# Autodesk Inventor assembly: artschallenge2022
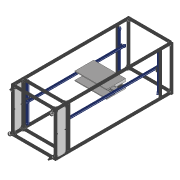
[picture p0: Inventor's stored thumbnail of the model, 180x180]
Saved by Autodesk Inventor 2020 (Build 240168000, 168)
## iProperties
Created: 2021-10-24
Part Number: artschallenge2022
Description: CAx-IF Rec.Pracs.---Model Styling and Organization---1.2---2011-12-15
Document SubType Name: Assembly
Designer: ken113
Sending System: 3D_Kernel_IO2017 Sp2 by CT CoreTechnologie
Preprocessor: STEP Interface 2017 Sp2 by CT CoreTechnologie
Title: artschallenge2022.stp
## Documents named in this file (61)
- D:\Document\Github\Eto_Project\Hardware\Parts\MISUMI_FRAMES\model_ver2\artschallenge2022.iam
- D:\Document\Github\Eto_Project\Hardware\Parts\MISUMI_FRAMES\model_ver2\NEFSB8-4040-200.ipt
- D:\Document\Github\Eto_Project\Hardware\Parts\MISUMI_FRAMES\model_ver2\NEFSB8-4040-1030.ipt
- D:\Document\Github\Eto_Project\Hardware\Parts\MISUMI_FRAMES\model_ver2\NEFSB8-4040-950.ipt
- D:\Document\Github\Eto_Project\Hardware\Parts\MISUMI_FRAMES\model_ver2\HBLFSNB8-C-SET(1).iam
- D:\Document\Github\Eto_Project\Hardware\Parts\MISUMI_FRAMES\model_ver2\HBLFSNB8-C-SET(2).iam
- D:\Document\Github\Eto_Project\Hardware\Parts\MISUMI_FRAMES\model_ver2\HBLFSNB8-C-SET(3).iam
- D:\Document\Github\Eto_Project\Hardware\Parts\MISUMI_FRAMES\model_ver2\HBLFSNB8-C-SET(4).iam
- D:\Document\Github\Eto_Project\Hardware\Parts\MISUMI_FRAMES\model_ver2\HBLFSNB8-SET(1).iam
- D:\Document\Github\Eto_Project\Hardware\Parts\MISUMI_FRAMES\model_ver2\HBLFSNB8-SET(2).iam
- D:\Document\Github\Eto_Project\Hardware\Parts\MISUMI_FRAMES\model_ver2\HBLFSNB8-SET(3).iam
- D:\Document\Github\Eto_Project\Hardware\Parts\MISUMI_FRAMES\model_ver2\HBLFSNB8-SET(4).iam
- D:\Document\Github\Eto_Project\Hardware\Parts\MISUMI_FRAMES\model_ver2\HBLFSNB8-SET(5).iam
- D:\Document\Github\Eto_Project\Hardware\Parts\MISUMI_FRAMES\model_ver2\HBLFSNB8-SET(6).iam
- D:\Document\Github\Eto_Project\Hardware\Parts\MISUMI_FRAMES\model_ver2\HBLFSNB8-SET(7).iam
- D:\Document\Github\Eto_Project\Hardware\Parts\MISUMI_FRAMES\model_ver2\HBLFSNB8-SET(8).iam
- D:\Document\Github\Eto_Project\Hardware\Parts\MISUMI_FRAMES\model_ver2\HBLFSNB8-C-SET(5).iam
- D:\Document\Github\Eto_Project\Hardware\Parts\MISUMI_FRAMES\model_ver2\HBLFSNB8-C-SET(6).iam
- D:\Document\Github\Eto_Project\Hardware\Parts\MISUMI_FRAMES\model_ver2\HBLFSNB8-SET(9).iam
- D:\Document\Github\Eto_Project\Hardware\Parts\MISUMI_FRAMES\model_ver2\HBLFSNB8-SET(10).iam
- D:\Document\Github\Eto_Project\Hardware\Parts\MISUMI_FRAMES\model_ver2\HBLFSNB8-SET(11).iam
- D:\Document\Github\Eto_Project\Hardware\Parts\MISUMI_FRAMES\model_ver2\HBLFSNB8-SET(12).iam
- D:\Document\Github\Eto_Project\Hardware\Parts\MISUMI_FRAMES\model_ver2\HBLFSNB8-SET(13).iam
- D:\Document\Github\Eto_Project\Hardware\Parts\MISUMI_FRAMES\model_ver2\HBLFSNB8-SET(14).iam
- D:\Document\Github\Eto_Project\Hardware\Parts\MISUMI_FRAMES\model_ver2\HBLFSNB8-SET(15).iam
- D:\Document\Github\Eto_Project\Hardware\Parts\MISUMI_FRAMES\model_ver2\HBLFSNB8-SET(16).iam
- D:\Document\Github\Eto_Project\Hardware\Parts\MISUMI_FRAMES\model_ver2\HBLFSNB8-C-SET(7).iam
- D:\Document\Github\Eto_Project\Hardware\Parts\MISUMI_FRAMES\model_ver2\HBLFSNB8-C-SET(8).iam
- D:\Document\Github\Eto_Project\Hardware\Parts\MISUMI_FRAMES\model_ver2\NEFSB8-4040-2400.ipt
- D:\Document\Github\Eto_Project\Hardware\Parts\MISUMI_FRAMES\model_ver2\ACBA6H-948-198-3-F463-G176-N5.ipt
- D:\Document\Github\Eto_Project\Hardware\Parts\MISUMI_FRAMES\model_ver2\HSMCS75-R.iam
- D:\Document\Github\Eto_Project\Hardware\Parts\MISUMI_FRAMES\model_ver2\HBLFSNB8-SET(17).iam
- D:\Document\Github\Eto_Project\Hardware\Parts\MISUMI_FRAMES\model_ver2\HBLFSNB8-SET(18).iam
- D:\Document\Github\Eto_Project\Hardware\Parts\MISUMI_FRAMES\model_ver2\HBLFSNB8-SET(19).iam
- D:\Document\Github\Eto_Project\Hardware\Parts\MISUMI_FRAMES\model_ver2\HBLFSNB8-SET(20).iam
- D:\Document\Github\Eto_Project\Hardware\Parts\MISUMI_FRAMES\model_ver2\HBLFSNB8-SET(21).iam
- D:\Document\Github\Eto_Project\Hardware\Parts\MISUMI_FRAMES\model_ver2\HBLFSNB8-SET(22).iam
- D:\Document\Github\Eto_Project\Hardware\Parts\MISUMI_FRAMES\model_ver2\HBLFSNB8-SET(23).iam
- D:\Document\Github\Eto_Project\Hardware\Parts\MISUMI_FRAMES\model_ver2\HBLFSNB8-SET(24).iam
- D:\Document\Github\Eto_Project\Hardware\Parts\MISUMI_FRAMES\model_ver2\HBLFSNB8-SET(25).iam
- D:\Document\Github\Eto_Project\Hardware\Parts\MISUMI_FRAMES\model_ver2\HBLFSNB8-SET(26).iam
- D:\Document\Github\Eto_Project\Hardware\Parts\MISUMI_FRAMES\model_ver2\HBLFSNB8-SET(27).iam
- D:\Document\Github\Eto_Project\Hardware\Parts\MISUMI_FRAMES\model_ver2\HBLFSNB8-SET(28).iam
- D:\Document\Github\Eto_Project\Hardware\Parts\MISUMI_FRAMES\model_ver2\HBLFSNB8-SET(29).iam
- D:\Document\Github\Eto_Project\Hardware\Parts\MISUMI_FRAMES\model_ver2\HBLFSNB8-SET(30).iam
- D:\Document\Github\Eto_Project\Hardware\Parts\MISUMI_FRAMES\model_ver2\HBLFSNB8-SET(31).iam
- D:\Document\Github\Eto_Project\Hardware\Parts\MISUMI_FRAMES\model_ver2\HBLFSNB8-SET(32).iam
- D:\Document\Github\Eto_Project\Hardware\Parts\MISUMI_FRAMES\model_ver2\HBLFSNB8-SET(33).iam
- D:\Document\Github\Eto_Project\Hardware\Parts\MISUMI_FRAMES\model_ver2\HBLFSNB8-SET(34).iam
- D:\Document\Github\Eto_Project\Hardware\Parts\MISUMI_FRAMES\model_ver2\HBLFSNB8-SET(35).iam
- D:\Document\Github\Eto_Project\Hardware\Parts\MISUMI_FRAMES\model_ver2\HBLFSNB8-SET(36).iam
- D:\Document\Github\Eto_Project\Hardware\Parts\MISUMI_FRAMES\model_ver2\HCBM5-8.ipt
- D:\Document\Github\Eto_Project\Hardware\Parts\MISUMI_FRAMES\model_ver2\HCBR8.ipt
- D:\Document\Github\Eto_Project\Hardware\Parts\MISUMI_FRAMES\model_ver2\HNTT8-8.ipt
- D:\Document\Github\Eto_Project\Hardware\Parts\MISUMI_FRAMES\model_ver2\CBM8-12.ipt
- D:\Document\Github\Eto_Project\Hardware\Parts\MISUMI_FRAMES\model_ver2\HCBM5-15.ipt
- D:\Document\Github\Eto_Project\Hardware\Parts\CCM\CCM motion linear guide rail\CCM_UNIT\CCM_Unit_A.iam
- D:\Document\Github\Eto_Project\Hardware\Parts\CCM\CCM motion linear guide rail\CCM_UNIT\CCM_Unit_B.iam
- D:\Document\Github\Eto_Project\Hardware\Parts\CCM\CCM motion linear guide rail\CCM_UNIT\CCM_Unit_C.iam
- D:\Document\Github\Eto_Project\Hardware\Parts\CCM\CCM motion linear guide rail\CCM_UNIT\CCM_Unit_D.iam
- D:\Document\Github\Eto_Project\Hardware\Parts\Display\Display_A.ipt
## Components (130 placed, 60 different names)
1. NEFSB8-4040-200
2. NEFSB8-4040-200:1
3. NEFSB8-4040-200:2
4. NEFSB8-4040-200:3
5. NEFSB8-4040-1030
6. NEFSB8-4040-1030:1 — メイト:4, メイト:5
7. NEFSB8-4040-950
8. NEFSB8-4040-950:1
9. HBLFSNB8-C-SET(1) [sub-assembly]
10. HBLFSNB8-C-SET(2) [sub-assembly]
11. HBLFSNB8-C-SET(3) [sub-assembly]
12. HBLFSNB8-C-SET(4) [sub-assembly]
13. HBLFSNB8-SET(1) [sub-assembly]
14. HBLFSNB8-SET(2) [sub-assembly]
15. HBLFSNB8-SET(3) [sub-assembly]
16. HBLFSNB8-SET(4) [sub-assembly]
17. HBLFSNB8-SET(5) [sub-assembly]
18. HBLFSNB8-SET(6) [sub-assembly]
19. HBLFSNB8-SET(7) [sub-assembly]
20. HBLFSNB8-SET(8) [sub-assembly]
21. NEFSB8-4040-1030:2
22. NEFSB8-4040-950:2
23. NEFSB8-4040-950:3
24. NEFSB8-4040-1030:3
25. HBLFSNB8-C-SET(5) [sub-assembly]
26. HBLFSNB8-C-SET(6) [sub-assembly]
27. HBLFSNB8-SET(9) [sub-assembly]
28. HBLFSNB8-SET(10) [sub-assembly]
29. HBLFSNB8-SET(11) [sub-assembly]
30. HBLFSNB8-SET(12) [sub-assembly]
31. HBLFSNB8-SET(13) [sub-assembly]
32. HBLFSNB8-SET(14) [sub-assembly]
33. HBLFSNB8-SET(15) [sub-assembly]
34. HBLFSNB8-SET(16) [sub-assembly]
35. HBLFSNB8-C-SET(7) [sub-assembly]
36. HBLFSNB8-C-SET(8) [sub-assembly]
37. NEFSB8-4040-2400 — メイト:2, メイト:15, フラッシュ:17, メイト:16, フラッシュ:19
38. NEFSB8-4040-2400:1 — 角度:2, メイト:3
39. NEFSB8-4040-2400:2 — 角度:1, メイト:1, メイト:6, メイト:13, フラッシュ:14, メイト:14
40. NEFSB8-4040-2400:3 — 角度:3
41. NEFSB8-4040-1030:4
42. NEFSB8-4040-1030:5 — 角度:4
43. ACBA6H-948-198-3-F463-G176-N5
44. ACBA6H-948-198-3-F463-G176-N5:1
45. HSMCS75-R [sub-assembly]
46. HSMCS75-R:1 [sub-assembly]
47. HSMCS75-R:2 [sub-assembly]
48. HSMCS75-R:3 [sub-assembly]
49. HBLFSNB8-SET(17) [sub-assembly]
50. HBLFSNB8-SET(18) [sub-assembly]
51. HBLFSNB8-SET(19) [sub-assembly]
52. HBLFSNB8-SET(20) [sub-assembly]
53. HBLFSNB8-SET(21) [sub-assembly]
54. HBLFSNB8-SET(22) [sub-assembly]
55. HBLFSNB8-SET(23) [sub-assembly]
56. HBLFSNB8-SET(24) [sub-assembly]
57. HBLFSNB8-SET(25) [sub-assembly]
58. HBLFSNB8-SET(26) [sub-assembly]
59. HBLFSNB8-SET(27) [sub-assembly]
60. HBLFSNB8-SET(28) [sub-assembly]
61. HBLFSNB8-SET(29) [sub-assembly]
62. HBLFSNB8-SET(30) [sub-assembly]
63. HBLFSNB8-SET(31) [sub-assembly]
64. HBLFSNB8-SET(32) [sub-assembly]
65. HBLFSNB8-SET(33) [sub-assembly]
66. HBLFSNB8-SET(34) [sub-assembly]
67. HBLFSNB8-SET(35) [sub-assembly]
68. HBLFSNB8-SET(36) [sub-assembly]
69. NEFSB8-4040-950:4
70. NEFSB8-4040-950:5
71. HCBM5-8
72. HCBM5-8:1
73. HCBM5-8:2
74. HCBM5-8:3
75. HCBR8
76. HCBR8:1
77. HCBM5-8:4
78. HCBM5-8:5
79. HCBM5-8:6
80. HCBM5-8:7
81. HCBR8:2
82. HCBR8:3
83. HNTT8-8
84. CBM8-12
85. HNTT8-8:1
86. CBM8-12:1
87. HNTT8-8:2
88. CBM8-12:2
89. HNTT8-8:3
90. CBM8-12:3
91. HNTT8-8:4
92. CBM8-12:4
93. HNTT8-8:5
94. CBM8-12:5
95. HNTT8-8:6
96. CBM8-12:6
97. HNTT8-8:7
98. CBM8-12:7
99. HNTT8-8:8
100. CBM8-12:8
101. HNTT8-8:9
102. CBM8-12:9
103. HNTT8-8:10
104. CBM8-12:10
105. HNTT8-8:11
106. CBM8-12:11
107. HNTT8-8:12
108. CBM8-12:12
109. HNTT8-8:13
110. CBM8-12:13
111. HNTT8-8:14
112. CBM8-12:14
113. HNTT8-8:15
114. CBM8-12:15
115. HCBM5-15
116. HCBM5-15:1
117. HCBM5-15:2
118. HCBM5-15:3
119. CCM_Unit_A:1 [sub-assembly] — 角度:2, フラッシュ:1, フラッシュ:2, メイト:7, メイト:8, フラッシュ:8, メイト:9, フラッシュ:10, メイト:12, メイト:17
120. CCM_Unit_B:1 [sub-assembly] — 角度:1, 角度:3, フラッシュ:1, フラッシュ:2, メイト:10, フラッシュ:10, メイト:11, フラッシュ:12
121. CCM_Unit_C:1 [sub-assembly] — メイト:1, フラッシュ:3, フラッシュ:5, メイト:6, フラッシュ:6, メイト:9, フラッシュ:16
122. CCM_Unit_C:2 [sub-assembly] — メイト:2, 角度:4, フラッシュ:4, フラッシュ:7, フラッシュ:9, メイト:10
123. CCM_Unit_D:1 [sub-assembly] — メイト:4, フラッシュ:3, フラッシュ:5, メイト:5
124. CCM_Unit_D:2 [sub-assembly] — メイト:3, フラッシュ:4, フラッシュ:6, フラッシュ:7, メイト:7, メイト:8, フラッシュ:8, フラッシュ:9, フラッシュ:15
125. Display_A:1 — 角度:5, フラッシュ:11, メイト:11, フラッシュ:13
126. Display_A:2 — 角度:5, フラッシュ:11, メイト:12, フラッシュ:12, フラッシュ:13, メイト:17
127. NEFSB8-4040-950:7 — メイト:13, フラッシュ:14, フラッシュ:15, フラッシュ:20
128. NEFSB8-4040-950:8 — メイト:16, フラッシュ:19, フラッシュ:20
129. NEFSB8-4040-950:9 — メイト:15, フラッシュ:17, フラッシュ:18
130. NEFSB8-4040-950:10 — メイト:14, フラッシュ:16, フラッシュ:18
## Relationships (42: Flush 20, Mate 17, Angle 5)
- 角度:1 [Angle] (0 deg): NEFSB8-4040-2400:2 ↔ CCM_Unit_B:1
- 角度:2 [Angle] (180 deg): NEFSB8-4040-2400:1 ↔ CCM_Unit_A:1
- 角度:3 [Angle] (0 deg): NEFSB8-4040-2400:3 ↔ CCM_Unit_B:1
- フラッシュ:1 [Flush]: CCM_Unit_A:1 ↔ CCM_Unit_B:1
- フラッシュ:2 [Flush]: CCM_Unit_A:1 ↔ CCM_Unit_B:1
- メイト:1 [Mate] (2 mm): NEFSB8-4040-2400:2 ↔ CCM_Unit_C:1
- メイト:2 [Mate] (2 mm): NEFSB8-4040-2400 ↔ CCM_Unit_C:2
- 角度:4 [Angle] (0 deg): NEFSB8-4040-1030:5 ↔ CCM_Unit_C:2
- メイト:3 [Mate] (2 mm): NEFSB8-4040-2400:1 ↔ CCM_Unit_D:2
- メイト:4 [Mate] (2 mm): NEFSB8-4040-1030:1 ↔ CCM_Unit_D:1
- フラッシュ:3 [Flush]: CCM_Unit_C:1 ↔ CCM_Unit_D:1
- フラッシュ:4 [Flush]: CCM_Unit_C:2 ↔ CCM_Unit_D:2
- フラッシュ:5 [Flush]: CCM_Unit_C:1 ↔ CCM_Unit_D:1
- メイト:5 [Mate] (20 mm): NEFSB8-4040-1030:1 ↔ CCM_Unit_D:1
- メイト:6 [Mate] (50 mm): NEFSB8-4040-2400:2 ↔ CCM_Unit_C:1
- フラッシュ:6 [Flush]: CCM_Unit_C:1 ↔ CCM_Unit_D:2
- フラッシュ:7 [Flush]: CCM_Unit_C:2 ↔ CCM_Unit_D:2
- メイト:7 [Mate]: CCM_Unit_A:1 ↔ CCM_Unit_D:2
- メイト:8 [Mate] (2 mm): CCM_Unit_A:1 ↔ CCM_Unit_D:2
- フラッシュ:8 [Flush] (20 mm): CCM_Unit_A:1 ↔ CCM_Unit_D:2
- メイト:9 [Mate]: CCM_Unit_A:1 ↔ CCM_Unit_C:1
- フラッシュ:9 [Flush]: CCM_Unit_C:2 ↔ CCM_Unit_D:2
- メイト:10 [Mate] (2 mm): CCM_Unit_B:1 ↔ CCM_Unit_C:2
- フラッシュ:10 [Flush]: CCM_Unit_A:1 ↔ CCM_Unit_B:1
- 角度:5 [Angle] (180 deg): Display_A:1 ↔ Display_A:2
- フラッシュ:11 [Flush]: Display_A:1 ↔ Display_A:2
- メイト:11 [Mate] (5 mm): CCM_Unit_B:1 ↔ Display_A:1
- メイト:12 [Mate] (5 mm): CCM_Unit_A:1 ↔ Display_A:2
- フラッシュ:12 [Flush] (-100 mm): CCM_Unit_B:1 ↔ Display_A:2
- フラッシュ:13 [Flush]: Display_A:1 ↔ Display_A:2
- メイト:13 [Mate]: NEFSB8-4040-2400:2 ↔ NEFSB8-4040-950:7
- フラッシュ:14 [Flush]: NEFSB8-4040-2400:2 ↔ NEFSB8-4040-950:7
- フラッシュ:15 [Flush]: CCM_Unit_D:2 ↔ NEFSB8-4040-950:7
- メイト:14 [Mate]: NEFSB8-4040-2400:2 ↔ NEFSB8-4040-950:10
- フラッシュ:16 [Flush]: CCM_Unit_C:1 ↔ NEFSB8-4040-950:10
- メイト:15 [Mate]: NEFSB8-4040-2400 ↔ NEFSB8-4040-950:9
- フラッシュ:17 [Flush]: NEFSB8-4040-2400 ↔ NEFSB8-4040-950:9
- フラッシュ:18 [Flush]: NEFSB8-4040-950:9 ↔ NEFSB8-4040-950:10
- メイト:16 [Mate]: NEFSB8-4040-2400 ↔ NEFSB8-4040-950:8
- フラッシュ:19 [Flush]: NEFSB8-4040-2400 ↔ NEFSB8-4040-950:8
- フラッシュ:20 [Flush]: NEFSB8-4040-950:7 ↔ NEFSB8-4040-950:8
- メイト:17 [Mate] (4 mm): CCM_Unit_A:1 ↔ Display_A:2
